# Autodesk Inventor assembly: Motor_assembly
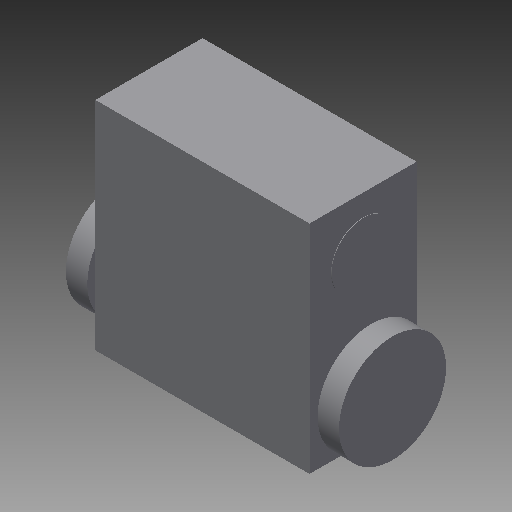
[picture p0: Inventor's stored thumbnail of the model, 512x512]
Saved by Autodesk Inventor 2019 (Build 230136000, 136)
## iProperties
Created: 2019-02-07
Part Number: Motor_assembly
Document SubType Name: Assembly
Designer: USUARIO
Author: USUARIO
## Documents named in this file (3)
- D:\Users\Documents\Inventor parts\Structure_Charlotte\Structure_Charlotte\Motor_assembly.iam
- D:\Users\Documents\Inventor parts\Structure_Charlotte\Structure_Charlotte\Motor.ipt
- D:\Users\Documents\Inventor parts\Structure_Charlotte\Structure_Charlotte\Motor_joint.ipt
## Components (3 placed, 2 different names)
1. Motor:1 — Mate:3, Rotational:3, Mate:4, Rotational:4
2. Motor_joint:2 — Mate:4, Rotational:4
3. Motor_joint:3 — Mate:3, Rotational:3
## Relationships (4: Mate 2, RevoluteJoint 2)
- Mate:3: Motor:1 ↔ Motor_joint:3
- Rotational:3 [RevoluteJoint]: Motor:1 ↔ Motor_joint:3
- Mate:4: Motor:1 ↔ Motor_joint:2
- Rotational:4 [RevoluteJoint]: Motor:1 ↔ Motor_joint:2
